# Autodesk Inventor assembly: Assembly1
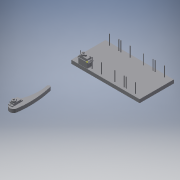
[picture p0: Inventor's stored thumbnail of the model, 180x180]
Saved by Autodesk Inventor 2018 (Build 220112000, 112)
## iProperties
Created: 2017-12-28
Part Number: Assembly1
Document SubType Name: Assembly
Designer: BB-8
Author: BB-8
## Documents named in this file (5)
- C:\Users\BB-8\Desktop\asimov\leg\Assembly1.iam
- C:\Users\BB-8\Desktop\asimov\servopocket.ipt
- C:\Users\BB-8\Desktop\asimov\sg90.ipt
- C:\Users\BB-8\Desktop\asimov\leg\leg.ipt
- C:\Users\BB-8\Desktop\asimov\leg\Part4.ipt
## Components (5 placed, 4 different names)
1. servopocket:1 — Mate:1, Mate:2, Mate:3
2. sg90:1 — Mate:1, Mate:2, Mate:3, Mate:7, Mate:8, Mate:9
3. leg:1 — Mate:4, Mate:5, Mate:6
4. sg90:2 — Mate:4, Mate:5, Mate:6
5. Part4:1 — Mate:7, Mate:8, Mate:9
## Relationships (9: Mate 9)
- Mate:1: servopocket:1 ↔ sg90:1
- Mate:2: servopocket:1 ↔ sg90:1
- Mate:3: servopocket:1 ↔ sg90:1
- Mate:4: leg:1 ↔ sg90:2
- Mate:5: leg:1 ↔ sg90:2
- Mate:6: leg:1 ↔ sg90:2
- Mate:7: sg90:1 ↔ Part4:1
- Mate:8: sg90:1 ↔ Part4:1
- Mate:9: sg90:1 ↔ Part4:1
